# Autodesk Inventor assembly: hang support
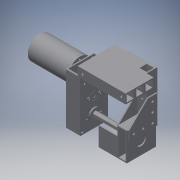
[picture p0: Inventor's stored thumbnail of the model, 180x180]
Saved by Autodesk Inventor 2016 (Build 200138000, 138)
## iProperties
Created: 2016-04-20
Part Number: hang support
Document SubType Name: Assembly
Designer: gus
Author: gus
## Documents named in this file (8)
- \\Mac\Home\Desktop\1510-stronghold-CAD-master\hang arm 2.0\hang support.iam
- \\Mac\Home\Desktop\1510-stronghold-CAD-master\hang arm 2.0\support block.ipt
- \\Mac\Home\Desktop\1510-stronghold-CAD-master\hang arm 2.0\support block 2.ipt
- \\Mac\Home\Desktop\1510-stronghold-CAD-master\hang arm 2.0\upright beam.ipt
- \\Mac\Home\Desktop\1510-stronghold-CAD-master\hang arm 2.0\gusset.ipt
- \\Mac\Home\Desktop\1510-stronghold-CAD-master\hang arm 2.0\other end support.ipt
- \\Mac\Home\Desktop\1510-stronghold-CAD-master\hang arm 2.0\angle gusset.ipt
- \\Mac\Home\Desktop\1510-stronghold-CAD-master\hang arm 2.0\tb nano\Toughbox+Nano+All+Shafts+v2-2.ipt
## Components (11 placed, 7 different names)
1. support block:2 — Flush:3, Flush:4, Flush:5, Flush:6, Flush:7, Flush:8, Flush:13, Flush:14, Mate:4
2. support block:3 — Flush:3, Flush:4, Mate:5
3. support block 2:1 — Flush:5, Flush:6, Flush:7, Flush:9, Mate:3, Flush:11
4. upright beam:1 — Flush:8, Flush:9, Mate:3, Flush:10, Flush:12, Flush:16, Flush:25, Mate:6, Flush:26, Mate:8, Flush:28
5. gusset:1 — Flush:10, Flush:11, Flush:12
6. support block:4 — Flush:13, Flush:14, Mate:4, Mate:5
7. other end support:1 — Flush:16, Flush:20, Flush:23, Flush:24, Flush:25, Mate:6, Mate:7, Flush:27, Flush:29, Flush:30
8. angle gusset:1 — Flush:20, Flush:21, Flush:23, Flush:24
9. Toughbox+Nano+All+Shafts+v2-2:1 — Flush:21, Flush:30
10. gusset:2 — Mate:7, Flush:26, Flush:27
11. gusset:3 — Mate:8, Flush:28, Flush:29
## Relationships (29: Flush 23, Mate 6)
- Flush:3: support block:2 ↔ support block:3
- Flush:4: support block:2 ↔ support block:3
- Flush:5: support block:2 ↔ support block 2:1
- Flush:6: support block:2 ↔ support block 2:1
- Flush:7: support block:2 ↔ support block 2:1
- Flush:8: support block:2 ↔ upright beam:1
- Flush:9: support block 2:1 ↔ upright beam:1
- Mate:3: support block 2:1 ↔ upright beam:1
- Flush:10: upright beam:1 ↔ gusset:1
- Flush:11: support block 2:1 ↔ gusset:1
- Flush:12: upright beam:1 ↔ gusset:1
- Flush:13: support block:2 ↔ support block:4
- Flush:14: support block:2 ↔ support block:4
- Mate:4: support block:2 ↔ support block:4
- Mate:5: support block:3 ↔ support block:4
- Flush:16: upright beam:1 ↔ other end support:1
- Flush:20: other end support:1 ↔ angle gusset:1
- Flush:21: angle gusset:1 ↔ Toughbox+Nano+All+Shafts+v2-2:1
- Flush:23: other end support:1 ↔ angle gusset:1
- Flush:24: other end support:1 ↔ angle gusset:1
- Flush:25: upright beam:1 ↔ other end support:1
- Mate:6: upright beam:1 ↔ other end support:1
- Mate:7: other end support:1 ↔ gusset:2
- Flush:26: upright beam:1 ↔ gusset:2
- Flush:27 (50.8 mm): other end support:1 ↔ gusset:2
- Mate:8: upright beam:1 ↔ gusset:3
- Flush:28: upright beam:1 ↔ gusset:3
- Flush:29 (50.8 mm): other end support:1 ↔ gusset:3
- Flush:30: other end support:1 ↔ Toughbox+Nano+All+Shafts+v2-2:1
